# Autodesk Inventor assembly: servoArmsAssembly
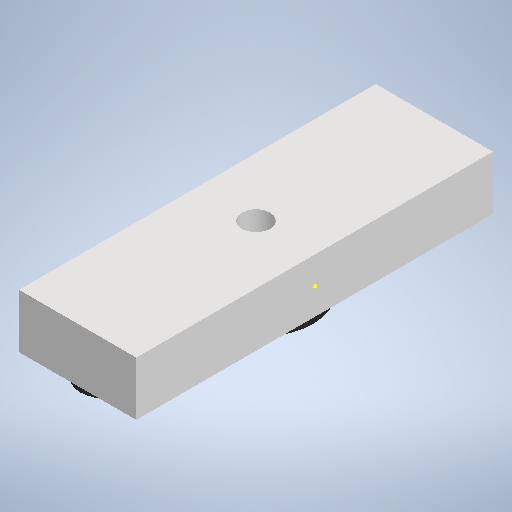
[picture p0: Inventor's stored thumbnail of the model, 512x512]
Saved by Autodesk Inventor 2025.1 (Build 291241020, 241B)
## iProperties
Created: 2024-09-10
Part Number: servoArmsAssembly
Document SubType Name: Assembly
Designer: omiye
Author: omiye
## Documents named in this file (3)
- C:\Projects\Arduino\hexapod\legModels\miscStuff\servoArmsAssembly.iam
- C:\Projects\Arduino\hexapod\legModels\straightServoHorn.ipt
- C:\Projects\Arduino\hexapod\legModels\miscStuff\servoArm.ipt
## Components (2 placed, 2 different names)
1. straightServoHorn:1 — Mate:1, Mate:2
2. servoArm:1 — Mate:1, Mate:2, Mate:3
## Relationships (3: Mate 3)
- Mate:1: straightServoHorn:1 ↔ servoArm:1
- Mate:2: straightServoHorn:1 ↔ servoArm:1
- Mate:3: servoArm:1
